# Autodesk Inventor assembly: Assembly1
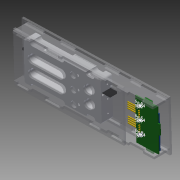
[picture p0: Inventor's stored thumbnail of the model, 180x180]
Saved by Autodesk Inventor 2015 (Build 190159000, 159)
## iProperties
Created: 2015-06-16
Part Number: Assembly1
Document SubType Name: Assembly
Designer: Openlab
Author: Openlab
## Documents named in this file (12)
- C:\Users\Admin\Alexey\OSS-Spectrophotometer\parts\Assembly1.iam
- C:\Users\Admin\Alexey\OSS-Spectrophotometer\parts\Bottom_V3.ipt
- C:\Users\Admin\Alexey\OSS-Spectrophotometer\parts\Led_Board_V1.ipt
- C:\Users\Admin\Alexey\OSS-Spectrophotometer\parts\Sensor_Board_dummy.ipt
- C:\Users\Admin\Alexey\OSS-Spectrophotometer\parts\Top_V4.ipt
- C:\Users\Admin\Alexey\OSS-Spectrophotometer\parts\Top_plate2.ipt
- C:\Users\Admin\Alexey\OSS-Spectrophotometer\parts\Large_retainer.ipt
- C:\Users\Admin\Alexey\OSS-Spectrophotometer\parts\Bottom_plate2.ipt
- C:\Users\Admin\Alexey\OSS-Spectrophotometer\parts\Left_wall.ipt
- C:\Users\Admin\Alexey\OSS-Spectrophotometer\parts\Right_wall.ipt
- C:\Users\Admin\Alexey\OSS-Spectrophotometer\parts\Cuvette_retainer2.ipt
- C:\Users\Admin\Alexey\OSS-Spectrophotometer\parts\Motherboard_assembly.iam
## Components (12 placed, 11 different names)
1. Bottom_V3:1 — Mate:1, Mate:2, Mate:3, Mate:4, Mate:7, Mate:10, Mate:11, Mate:12, Mate:13, Mate:14, Mate:15, Mate:16, Mate:18, Mate:19, Mate:20, Mate:21, Mate:22
2. Led_Board_V1:1 — Mate:4, Mate:13, Mate:14
3. Sensor_Board_dummy:1 — Mate:7, Mate:15, Mate:16
4. Top_V4:1 — Mate:1, Mate:2, Mate:3, Mate:17
5. Top_plate2:1 — Mate:17, Mate:18, Mate:19, Mate:24, Mate:26, Mate:30, Mate:31, Mate:32, Mate:33
6. Large_retainer:1
7. Large_retainer:2
8. Bottom_plate2:1 — Mate:20, Mate:21, Mate:22
9. Left_wall:1 — Mate:24, Mate:26, Mate:30, Mate:35, Mate:36
10. Right_wall:1 — Mate:31, Mate:32, Mate:33, Mate:34
11. Cuvette_retainer2:1 — Mate:10, Mate:11, Mate:12
12. Motherboard_assembly:1 [sub-assembly] — Mate:34, Mate:35, Mate:36
## Relationships (27: Mate 27)
- Mate:1: Bottom_V3:1 ↔ Top_V4:1
- Mate:2: Bottom_V3:1 ↔ Top_V4:1
- Mate:3: Bottom_V3:1 ↔ Top_V4:1
- Mate:4: Bottom_V3:1 ↔ Led_Board_V1:1
- Mate:7: Bottom_V3:1 ↔ Sensor_Board_dummy:1
- Mate:10: Bottom_V3:1 ↔ Cuvette_retainer2:1
- Mate:11: Bottom_V3:1 ↔ Cuvette_retainer2:1
- Mate:12: Bottom_V3:1 ↔ Cuvette_retainer2:1
- Mate:13: Bottom_V3:1 ↔ Led_Board_V1:1
- Mate:14: Bottom_V3:1 ↔ Led_Board_V1:1
- Mate:15: Bottom_V3:1 ↔ Sensor_Board_dummy:1
- Mate:16: Bottom_V3:1 ↔ Sensor_Board_dummy:1
- Mate:17: Top_V4:1 ↔ Top_plate2:1
- Mate:18: Bottom_V3:1 ↔ Top_plate2:1
- Mate:19: Bottom_V3:1 ↔ Top_plate2:1
- Mate:20: Bottom_V3:1 ↔ Bottom_plate2:1
- Mate:21: Bottom_V3:1 ↔ Bottom_plate2:1
- Mate:22: Bottom_V3:1 ↔ Bottom_plate2:1
- Mate:24: Top_plate2:1 ↔ Left_wall:1
- Mate:26: Top_plate2:1 ↔ Left_wall:1
- Mate:30: Top_plate2:1 ↔ Left_wall:1
- Mate:31: Top_plate2:1 ↔ Right_wall:1
- Mate:32: Top_plate2:1 ↔ Right_wall:1
- Mate:33: Top_plate2:1 ↔ Right_wall:1
- Mate:34: Right_wall:1 ↔ Motherboard_assembly:1
- Mate:35: Left_wall:1 ↔ Motherboard_assembly:1
- Mate:36: Left_wall:1 ↔ Motherboard_assembly:1
